# Autodesk Inventor assembly: Existing_Basement_And_Transition
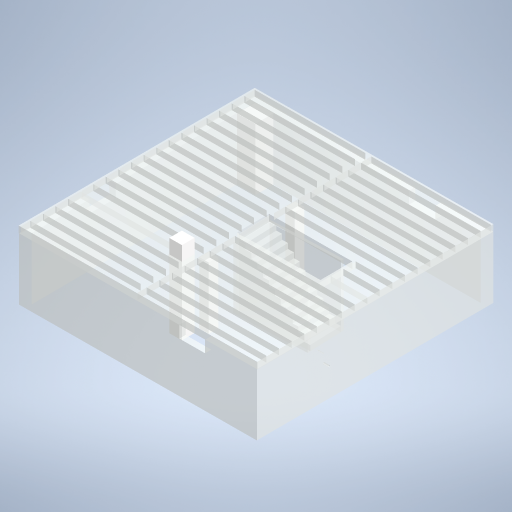
[picture p0: Inventor's stored thumbnail of the model, 512x512]
Saved by Autodesk Inventor 2024 (Build 280153000, 153)
## iProperties
Created: 2023-05-19
Part Number: Existing_Basement_And_Transition
Document SubType Name: Assembly
Designer: Tom
Author: Tom
## Documents named in this file (4)
- C:\Users\Tom\Documents\Tom_Levers_Public_Git_Repository\Inventor\Mobility\Existing_Basement_And_Existing_Basement_And_First_Floor_Transition.iam
- C:\Users\Tom\Documents\Tom_Levers_Public_Git_Repository\Inventor\Mobility\Basement\Existing_Basement.iam
- C:\Users\Tom\Documents\Tom_Levers_Public_Git_Repository\Inventor\Mobility\Existing_Basement_And_First_Floor_Transition.ipt
- C:\Users\Tom\Documents\Tom_Levers_Public_Git_Repository\Inventor\Mobility\Existing_Basement_And_Existing_Basement_And_First_Floor_Transition\AIP\FEA\ec90jbnb5.fres
## Components (2 placed, 2 different names)
1. Existing_Basement:1 [sub-assembly] — Mate:1, Flush:1, Flush:2
2. Existing_Basement_And_First_Floor_Transition:1 — Mate:1, Flush:1, Flush:2
## Relationships (3: Flush 2, Mate 1)
- Mate:1: Existing_Basement:1 ↔ Existing_Basement_And_First_Floor_Transition:1
- Flush:1: Existing_Basement:1 ↔ Existing_Basement_And_First_Floor_Transition:1
- Flush:2 (-215.9 mm): Existing_Basement:1 ↔ Existing_Basement_And_First_Floor_Transition:1
